# Autodesk Inventor assembly: robot
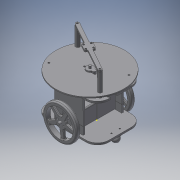
[picture p0: Inventor's stored thumbnail of the model, 180x180]
Saved by Autodesk Inventor 2017 (Build 210142000, 142)
## iProperties
Created: 2017-06-15
Part Number: robot
Document SubType Name: Assembly
Designer: millerid
Author: millerid
## Documents named in this file (14)
- U:\Research\Swarms\RobotModel\robot.iam
- U:\Research\Swarms\RobotModel\pcb.ipt
- U:\Research\Swarms\RobotModel\SG92R.ipt
- U:\Research\Swarms\RobotModel\NEMA11.ipt
- U:\Research\Swarms\RobotModel\halfincaster.ipt
- U:\Research\Swarms\RobotModel\1_5V_holder4AA.iam
- U:\Research\Swarms\RobotModel\Pololu 60mm Wheel.ipt
- U:\Research\Swarms\RobotModel\base_plate.ipt
- U:\Research\Swarms\RobotModel\top_plate.ipt
- U:\Research\Swarms\RobotModel\quarterin_spacer.ipt
- U:\Research\Swarms\RobotModel\led_brace.ipt
- U:\Research\Swarms\RobotModel\oneandquarterstandoff.ipt
- U:\Research\Swarms\RobotModel\side_plate_bottom.ipt
- U:\Research\Swarms\RobotModel\side_plate_top.ipt
## Components (22 placed, 13 different names)
1. pcb:1 — Mate:46, Mate:47, Mate:48, Mate:64, Mate:65, Mate:67, Mate:70, Mate:71, Mate:72, Mate:73, Mate:74
2. SG92R:1 — Mate:46, Mate:47, Mate:70
3. NEMA11:1 — Mate:3, Mate:82, Mate:83, Mate:84, Mate:89, Mate:90, Mate:91
4. NEMA11:2 — Mate:20, Mate:61, Mate:78, Mate:79, Mate:85, Mate:86, Mate:87, Mate:88
5. halfincaster:1 — Mate:56, Mate:57
6. 1_5V_holder4AA:1 [sub-assembly] — Mate:60, Mate:61
7. Pololu 60mm Wheel:1 — Mate:3
8. halfincaster:2 — Mate:54, Mate:55, Mate:75
9. base_plate:1 — Mate:51, Mate:52, Mate:53, Mate:54, Mate:55, Mate:56, Mate:57, Mate:60, Mate:75, Mate:76, Mate:77, Mate:80, Mate:81
10. Pololu 60mm Wheel:2 — Mate:20
11. top_plate:1 — Mate:62, Mate:63, Mate:66, Mate:68, Mate:69, Mate:92, Mate:93
12. led_brace:1 — Mate:36, Mate:37, Mate:38, Mate:40
13. oneandquarterstandoff:1 — Mate:36, Mate:37, Mate:74
14. oneandquarterstandoff:2 — Mate:38, Mate:40, Mate:48, Mate:73
15. quarterin_spacer:1 — Mate:62, Mate:63, Mate:64, Mate:65
16. quarterin_spacer:2 — Mate:69, Mate:72
17. quarterin_spacer:3 — Mate:66, Mate:67
18. quarterin_spacer:4 — Mate:68, Mate:71
19. side_plate_bottom:1 — Mate:76, Mate:77, Mate:78, Mate:79, Mate:85
20. side_plate_bottom:2 — Mate:80, Mate:81, Mate:82, Mate:83, Mate:84
21. side_plate_top:1 — Mate:86, Mate:87, Mate:88
22. side_plate_top:2 — Mate:89, Mate:90, Mate:91, Mate:92, Mate:93
## Relationships (50: Mate 50)
- Mate:3: NEMA11:1 ↔ Pololu 60mm Wheel:1
- Mate:20: NEMA11:2 ↔ Pololu 60mm Wheel:2
- Mate:36: led_brace:1 ↔ oneandquarterstandoff:1
- Mate:37: led_brace:1 ↔ oneandquarterstandoff:1
- Mate:38 (0.1 mm): led_brace:1 ↔ oneandquarterstandoff:2
- Mate:40: led_brace:1 ↔ oneandquarterstandoff:2
- Mate:46: pcb:1 ↔ SG92R:1
- Mate:47: pcb:1 ↔ SG92R:1
- Mate:48: pcb:1 ↔ oneandquarterstandoff:2
- Mate:51: base_plate:1
- Mate:52: base_plate:1
- Mate:53: base_plate:1
- Mate:54: halfincaster:2 ↔ base_plate:1
- Mate:55: halfincaster:2 ↔ base_plate:1
- Mate:56: halfincaster:1 ↔ base_plate:1
- Mate:57: halfincaster:1 ↔ base_plate:1
- Mate:60: 1_5V_holder4AA:1 ↔ base_plate:1
- Mate:61: NEMA11:2 ↔ 1_5V_holder4AA:1
- Mate:62: top_plate:1 ↔ quarterin_spacer:1
- Mate:63: top_plate:1 ↔ quarterin_spacer:1
- Mate:64: pcb:1 ↔ quarterin_spacer:1
- Mate:65: pcb:1 ↔ quarterin_spacer:1
- Mate:66: top_plate:1 ↔ quarterin_spacer:3
- Mate:67: pcb:1 ↔ quarterin_spacer:3
- Mate:68: top_plate:1 ↔ quarterin_spacer:4
- Mate:69: top_plate:1 ↔ quarterin_spacer:2
- Mate:70 (0.2 mm): pcb:1 ↔ SG92R:1
- Mate:71: pcb:1 ↔ quarterin_spacer:4
- Mate:72: pcb:1 ↔ quarterin_spacer:2
- Mate:73: pcb:1 ↔ oneandquarterstandoff:2
- Mate:74: pcb:1 ↔ oneandquarterstandoff:1
- Mate:75: halfincaster:2 ↔ base_plate:1
- Mate:76: base_plate:1 ↔ side_plate_bottom:1
- Mate:77: base_plate:1 ↔ side_plate_bottom:1
- Mate:78: NEMA11:2 ↔ side_plate_bottom:1
- Mate:79: NEMA11:2 ↔ side_plate_bottom:1
- Mate:80: base_plate:1 ↔ side_plate_bottom:2
- Mate:81: base_plate:1 ↔ side_plate_bottom:2
- Mate:82: NEMA11:1 ↔ side_plate_bottom:2
- Mate:83: NEMA11:1 ↔ side_plate_bottom:2
- Mate:84: NEMA11:1 ↔ side_plate_bottom:2
- Mate:85: NEMA11:2 ↔ side_plate_bottom:1
- Mate:86: NEMA11:2 ↔ side_plate_top:1
- Mate:87: NEMA11:2 ↔ side_plate_top:1
- Mate:88 (0.1 mm): NEMA11:2 ↔ side_plate_top:1
- Mate:89: NEMA11:1 ↔ side_plate_top:2
- Mate:90 (0.1 mm): NEMA11:1 ↔ side_plate_top:2
- Mate:91: NEMA11:1 ↔ side_plate_top:2
- Mate:92: top_plate:1 ↔ side_plate_top:2
- Mate:93: top_plate:1 ↔ side_plate_top:2
